# Autodesk Inventor assembly: 8098374 MS4-EM1FR-1/4-D6-E-P-M-AG-MPA-WPE-B
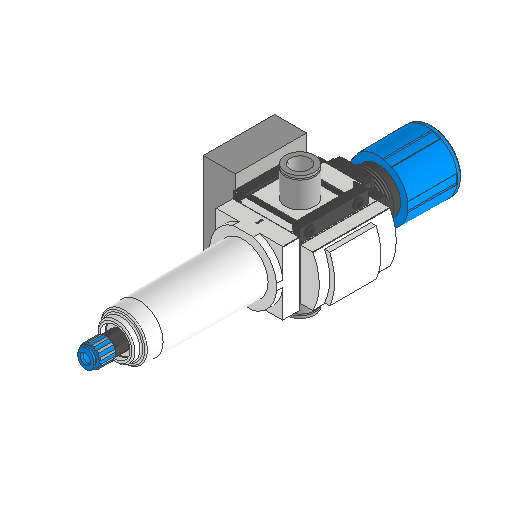
[picture p0: Inventor's stored thumbnail of the model, 512x512]
Saved by Autodesk Inventor 2024.3 (Build 283343000, 343)
## iProperties
Category: PARTsolutions
Company: FESTO
Created: 2025-04-26
Part Number: 8098374 MS4-EM1FR-1/4-D6-E-P-M-AG-MPA-WPE-B
Catalog Web Link: www.cadenas.de
Description: MSB4-Service unit combination
Vendor: FESTO
Document SubType Name: Assembly
Designer: psAdmin
Manufacturer: FESTO
Mass: 348.06 g
Surface Area: 648.208 cm^2
Volume: 367.834 cm^3
Density: 0.946243 g/cm^3
PSOL_IDENT_0: {$CADENAS_DATA/23d-libs/festo/parts/m/msb4/assemblies/msb4_cfg.prj},305 {VTYP=3D},{NB=8098374 MS4-EM
PSOL_IDENT_1: 1FR-1/4-D6-E-P-M-AG-MPA-WPE-B},{LINA=8098374 MS4-EM1FR-1/4-D6-E-P-M-AG-MPA-WPE-B},{NN=MSB4},{CNSFILE
PSOL_IDENT_2: NAME=8098374 MS4-EM1FR-1/4-D6-E-P-M-AG-MPA-WPE-B},{DATE=25.04.2025 18:07:15},{GEOMDATE=27.11.2024 07
PSOL_IDENT_3: :56:00},{VERSION=},{LINEID=10},{WBVAR=TYP,TNR,IDCODE,HIDE},{WBNUMERIC=HIDE}  {NB=8098374 MS4-EM1FR-1
PSOL_IDENT_4: /4-D6-E-P-M-AG-MPA-WPE-B},{LINA=8098374 MS4-EM1FR-1/4-D6-E-P-M-AG-MPA-WPE-B},{KT=DUMMY},{TYP=MSB4},{
PSOL_IDENT_5: TNR=8098374},{IDCODE=MS4-EM1FR-1/4-D6-E-P-M-AG-MPA-WPE-B},{HIDE=0}
NB: 8098374 MS4-EM1FR-1/4-D6-E-P-M-AG-MPA-WPE-B
NN: MSB4
NT: Service unit combination
NBSYN: $START@TNR. $START@IDCODE.
LINA: 8098374 MS4-EM1FR-1/4-D6-E-P-M-AG-MPA-WPE-B
CATALOG: Festo
TNR: 8098374
IDCODE: MS4-EM1FR-1/4-D6-E-P-M-AG-MPA-WPE-B
SUPPLIER: FESTO
ARTICLENO: 8098374 MS4-EM1FR-1/4-D6-E-P-M-AG-MPA-WPE-B
BOMINFO: 8098374 MS4-EM1FR-1/4-D6-E-P-M-AG-MPA-WPE-B
CREATOR: CADENAS GmbH
Title: 8098374 MS4-EM1FR-1/4-D6-E-P-M-AG-MPA-WPE-B
Author: Cadenas PARTsolutions
Comments: Service unit combination
## Documents named in this file (5)
- C:\MPA - shortPath\magisterka\V3\Workspace\Zakupowe\FESTO\MS4-EM1FR-14-D6-E-P-M-AG-MPA-WPE-B\8098374 MS4-EM1FR-1_4-D6-E-P-M-AG-MPA-WPE-B.iam
- C:\MPA - shortPath\magisterka\V3\Workspace\Zakupowe\FESTO\MS4-EM1FR-14-D6-E-P-M-AG-MPA-WPE-B\8098261 MS4-LFR-1_4-D6-E-P-M-AG-MPA-B---(high).ipt
- C:\MPA - shortPath\magisterka\V3\Workspace\Zakupowe\FESTO\MS4-EM1FR-14-D6-E-P-M-AG-MPA-WPE-B\8092760 MS4-MV-B---(46_high_m).ipt
- C:\MPA - shortPath\magisterka\V3\Workspace\Zakupowe\FESTO\MS4-EM1FR-14-D6-E-P-M-AG-MPA-WPE-B\8116179 MS4-MV-B---(0_high_m).ipt
- C:\MPA - shortPath\magisterka\V3\Workspace\Zakupowe\smc\KQ2S12-02AS_(A) Brass.ipt
## Components (5 placed, 4 different names)
1. 8098261 MS4-LFR-1_4-D6-E-P-M-AG-MPA-B---(high):1 — Insert:1, Insert:2
2. 8092760 MS4-MV-B---(46_high_m):1 — ANBAU_2_XY@3 <-> ANBAU_2_XY@4, ANBAU_2_Z@3 <-> ANBAU_2_Z@4, ANBAU_2_YZ@3 <-> ANBAU_2_YZ@4
3. 8116179 MS4-MV-B---(0_high_m):1 — ANBAU_2_XY@3 <-> ANBAU_2_XY@4, ANBAU_2_Z@3 <-> ANBAU_2_Z@4, ANBAU_2_YZ@3 <-> ANBAU_2_YZ@4
4. KQ2S12-02AS_(A) Brass:1 — Insert:2
5. KQ2S12-02AS_(A) Brass:2 — Insert:1
## Relationships (5: Mate 2, Insert 2, Angle 1)
- ANBAU_2_XY@3 <-> ANBAU_2_XY@4 [Mate]: 8092760 MS4-MV-B---(46_high_m):1 ↔ 8116179 MS4-MV-B---(0_high_m):1
- ANBAU_2_Z@3 <-> ANBAU_2_Z@4 [Mate]: 8092760 MS4-MV-B---(46_high_m):1 ↔ 8116179 MS4-MV-B---(0_high_m):1
- ANBAU_2_YZ@3 <-> ANBAU_2_YZ@4 [Angle] (180 deg): 8092760 MS4-MV-B---(46_high_m):1 ↔ 8116179 MS4-MV-B---(0_high_m):1
- Insert:1: 8098261 MS4-LFR-1_4-D6-E-P-M-AG-MPA-B---(high):1 ↔ KQ2S12-02AS_(A) Brass:2
- Insert:2: 8098261 MS4-LFR-1_4-D6-E-P-M-AG-MPA-B---(high):1 ↔ KQ2S12-02AS_(A) Brass:1
